# Autodesk Inventor assembly: Turn-Left-Right-Base
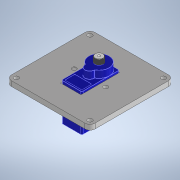
[picture p0: Inventor's stored thumbnail of the model, 180x180]
Saved by Autodesk Inventor 2022 (Build 260153000, 153)
## iProperties
Created: 2020-02-05
Part Number: Turn-Left-Right-Base
Document SubType Name: Assembly
Designer: joshn
Author: joshn
Revision Number: NONE
## Documents named in this file (5)
- D:\Joshwin Emmanuel\Fab_accad\git_hub\Fab_Work\arm\step\part\Turn-Left-Right-Base.iam
- D:\Joshwin Emmanuel\Fab_accad\git_hub\Fab_Work\arm\step\part\Pivot Servo Plate.ipt
- D:\Joshwin Emmanuel\Fab_accad\git_hub\Fab_Work\arm\step\part\Schraube _ Zylinder - M3,0 x 8,0.ipt
- D:\Joshwin Emmanuel\Fab_accad\git_hub\Fab_Work\arm\step\part\NONE_1.ipt
- D:\Joshwin Emmanuel\Fab_accad\git_hub\Fab_Work\arm\step\part\SG90 - Micro Servo 9g - Tower Pro.1.ipt
## Components (4 placed, 4 different names)
1. Pivot Servo Plate — Mate:1, Mate:2, Mate:3
2. Schraube : Zylinder - M3,0 x 8,0
3. Right Servo Tower Pro SG90 — Mate:1, Mate:2, Mate:3
4. Servo Retainer
## Relationships (3: Mate 3)
- Mate:1: Pivot Servo Plate ↔ Right Servo Tower Pro SG90
- Mate:2: Pivot Servo Plate ↔ Right Servo Tower Pro SG90
- Mate:3: Pivot Servo Plate ↔ Right Servo Tower Pro SG90
